# Autodesk Inventor assembly: Upper Arm
Saved by Autodesk Inventor 2014 SP1 (Build 180222100, 222)
## iProperties
Created: 2013-12-25
Part Number: Upper Arm
Document SubType Name: Assembly
Designer: tom
Author: tom
## Documents named in this file (3)
- C:\Users\tom\Documents\GitHub\Delta_Robots\Delatabot - Small Model\Imported Components\Deltabot - Small Model\Upper Arm.iam
- C:\Users\tom\Documents\GitHub\Delta_Robots\Delatabot - Small Model\Imported Components\Deltabot - Small Model\Component6.ipt
- C:\Users\tom\Documents\GitHub\Delta_Robots\Delatabot - Small Model\Imported Components\Deltabot - Small Model\Component7.ipt
## Components (2 placed, 2 different names)
1. Servo Hub 1
2. Servo Arm 1
## Relationships (3: Mate 3)
- [Mate]: Servo Hub 1 ↔ Servo Arm 1
- [Mate]: Servo Hub 1 ↔ Servo Arm 1
- [Mate]: Servo Hub 1 ↔ Servo Arm 1
